# Autodesk Inventor assembly: Demonstrator
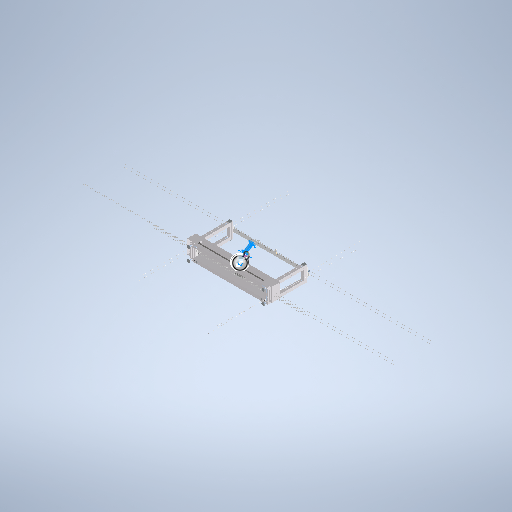
[picture p0: Inventor's stored thumbnail of the model, 512x512]
Saved by Autodesk Inventor 2025 (Build 290162010, 162A)
## iProperties
Created: 2024-11-07
Part Number: Demonstrator
Document SubType Name: Assembly
Designer: Admin
Mass: 19761.8 g
Surface Area: 23870.2 cm^2
Volume: 8041.77 cm^3
Density: 2.4574 g/cm^3
dummerWinkel: 1.5
Author: Admin
## Documents named in this file (25)
- C:\Users\Admin\GIT\HDVKBM\CAD\Krandemonstrator\Demonstrator.iam
- C:\Users\Admin\GIT\HDVKBM\CAD\Krandemonstrator\Träger.ipt
- C:\Users\Admin\Documents\Inventor\Content Center Files\R2025\de-DE\AS 1112 (2)\AS 1112 - M4  Typ 5.ipt
- C:\Users\Admin\GIT\HDVKBM\CAD\Krandemonstrator\MontageAufnahmeLO.ipt
- C:\Users\Admin\GIT\HDVKBM\CAD\Krandemonstrator\MontageAufnahmeLOV.ipt
- C:\Users\Admin\Documents\Inventor\Content Center Files\R2025\de-DE\AS 1427(03)\AS 1427 - M2 x 6(1).ipt
- C:\Users\Admin\GIT\HDVKBM\CAD\Krandemonstrator\Katze.iam
- C:\Users\Admin\GIT\HDVKBM\CAD\Krandemonstrator\UmlenkrolleHalterEinfach.iam
- C:\Users\Admin\GIT\HDVKBM\CAD\Krandemonstrator\SeilStange1m.ipt
- C:\Users\Admin\GIT\HDVKBM\CAD\Krandemonstrator\RollenhalterU.ipt
- C:\Users\Admin\GIT\HDVKBM\CAD\Krandemonstrator\UmlenkrolleHalterDoppelt.iam
- C:\Users\Admin\GIT\HDVKBM\CAD\Krandemonstrator\SeilatrappeHalter.ipt
- C:\Users\Admin\GIT\HDVKBM\CAD\Krandemonstrator\UmlenkrolleHalterDoppeltAngle.iam
- C:\Users\Admin\GIT\HDVKBM\CAD\Krandemonstrator\UmlenkrolleHalterEinfachAngle.iam
- C:\Users\Admin\GIT\HDVKBM\CAD\Krandemonstrator\UmlenkrolleHalterEinfachAngleB.iam
- C:\Users\Admin\GIT\HDVKBM\CAD\Krandemonstrator\seilatrappeHalterMini.ipt
- C:\Users\Admin\Documents\Inventor\Content Center Files\R2025\de-DE\AS 1421(4)\AS 1421 - M4 x 8 Kegelstumpf.ipt
- C:\Users\Admin\GIT\HDVKBM\CAD\Krandemonstrator\Schlitten.iam
- C:\Users\Admin\GIT\HDVKBM\CAD\Krandemonstrator\WS_10_40_930_2\WS_10_40_930_2.iam
- C:\Users\Admin\GIT\HDVKBM\CAD\Krandemonstrator\Frame.iam
- C:\Users\Admin\GIT\HDVKBM\CAD\Krandemonstrator\item_42006_nutenstein-8-st-m4-verzi__high\item_42006_nutenstein-8-st-m4-verzi__high.ipt
- C:\Users\Admin\Documents\Inventor\Content Center Files\R2025\de-DE\DIN 7991(2)\DIN 7991 - M4x30.ipt
- C:\Users\Admin\GIT\HDVKBM\CAD\Krandemonstrator\item_2623_nutenstein-8-st-m6-verzi__high\item_2623_nutenstein-8-st-m6-verzi__high.ipt
- C:\Users\Admin\Documents\Inventor\Content Center Files\R2025\de-DE\DIN 7991(2)\DIN 7991 - M6x16.ipt
- C:\Users\Admin\GIT\HDVKBM\CAD\Krandemonstrator\Zugfeder11.ipt
## Components (96 placed, 27 different names)
1. Katze:1 [sub-assembly] — KatzeLagerHO, KatzeLagerVV, KatzeSeilMutterVL, KatzeSeilMutterHL, KatzeSeilMutterVR, KatzeSeilMutterHR, KatzeGewindeSeilStumpfVL, KatzeGewindeSeilStumpfHL, KatzeGewindeSeilStumpfVR, KatzeGewindeSeilStumpfHR, KatzeSeilStumpfVL, KatzeSeilStumpfHL, KatzeSeilStumpfVR, KatzeSeilStumpfHR, Zylindrisch:83
2. Schlitten:1 [sub-assembly] — Verschiebbar:84, Zylindrisch:84, Zylindrisch:85, Zylindrisch:86, Zylindrisch:87, Planar:57, Planar:58, Planar:59, Planar:60
3. WS_10_40_930_2:1 [sub-assembly] — Zylindrisch:84, Zylindrisch:85, Zylindrisch:86, Zylindrisch:87, Starr:89, Starr:90, Starr:91, Starr:92, Starr:93, Starr:94, Starr:95, Starr:96, Starr:97
4. Frame:1 [sub-assembly] — Verschiebbar:85, Verschiebbar:86, Starr:83, Starr:88, Starr:89
5. item_42006_nutenstein-8-st-m4-verzi__high:1 — Starr:85
6. item_42006_nutenstein-8-st-m4-verzi__high:2 — Starr:84
7. item_42006_nutenstein-8-st-m4-verzi__high:3 — Starr:87
8. item_42006_nutenstein-8-st-m4-verzi__high:4 — Starr:86
9. DIN 7991 M4x30:1 — Passend:1
10. DIN 7991 M4x30:2 — Passend:2
11. DIN 7991 M4x30:3 — Passend:3
12. DIN 7991 M4x30:4 — Passend:4
13. DIN 7991 M6x16:1 — Starr:90, Starr:105
14. DIN 7991 M6x16:2 — Starr:91, Starr:104
15. DIN 7991 M6x16:3 — Starr:93, Starr:102
16. DIN 7991 M6x16:4 — Starr:92, Starr:103
17. DIN 7991 M6x16:5 — Starr:97, Starr:98
18. DIN 7991 M6x16:6 — Starr:96, Starr:99
19. DIN 7991 M6x16:7 — Starr:95, Starr:100
20. DIN 7991 M6x16:8 — Starr:94, Starr:101
21. item_2623_nutenstein-8-st-m6-verzi__high:1 — Starr:105
22. item_2623_nutenstein-8-st-m6-verzi__high:2 — Starr:104
23. item_2623_nutenstein-8-st-m6-verzi__high:3 — Starr:99
24. item_2623_nutenstein-8-st-m6-verzi__high:4 — Starr:103
25. item_2623_nutenstein-8-st-m6-verzi__high:5 — Starr:102
26. item_2623_nutenstein-8-st-m6-verzi__high:6 — Starr:101
27. item_2623_nutenstein-8-st-m6-verzi__high:7 — Starr:100
28. item_2623_nutenstein-8-st-m6-verzi__high:8 — Starr:98
29. Zugfeder1:1
30. MontageAufnahmeLOVV:2 — Starr:51, SeilrolleORHscrewA, SeilrolleORHscrewB, SeilrolleORHplan
31. MontageAufnahmeLO:2 — Starr:52, SeilrolleORVplan, SeilrolleORVscrewA, SeilrolleORVscrewB
32. MontageAufnahmeLOV:1 — SeilrolleOLVAuflage, SeilrolleOLVSchraubeA, SeilrolleOLVSchraubeB
33. MontageAufnahmeLOH:1 — SeilrolleOLHAuflage, SeilrolleOLHSchraubeA, SeilrolleOLHSchraubeB, Verschiebbar:85
34. Träger:1 — KatzeLagerHO, KatzeLagerVV, Starr:51, Starr:52, Verschiebbar:86
35. lastseil — Verschiebbar:84, Zylindrisch:83
36. seilatrappeHalterMini:3 — SeilAtrappeHalterMini3, SeilAtrappeHalterMini3Seil
37. seilatrappeHalterMini:4 — SeilAtrappeHalterMini4, SeilAtrappeHalterMini4Seil
38. SeilStange1m:16 — SeilrolleULMVsld, SeilAtrappeHalterMini3Seil, Planar:58
39. SeilStange1m:17 — SeilrolleULMHsld, SeilAtrappeHalterMini4Seil, Planar:57
40. SeilStange1m:18 — SeilAtrappeHalterMini1Seil, SeilrolleORVver, SeilrolleURMVver
41. SeilStange1m:19 — SeilAtrappeHalterMini2Seil, SeilrolleORHver, SeilrolleURMHver
42. seilatrappeHalterMini:1 — SeilAtrappeHalterMini1, SeilAtrappeHalterMini1Seil
43. seilatrappeHalterMini:2 — SeilAtrappeHalterMini2, SeilAtrappeHalterMini2Seil
44. SeilStange1m:13 — SeilrolleURHsld, Planar:59
45. SeilStange1m:12 — SeilrolleURVsld, Planar:60
46. SeilatrappeHalter:1 — SeilAtrappeHalterSeilA, SeilAtrappeHalterSeilB
47. SeilStange1m:1 — KatzeGewindeSeilStumpfVL, SeilrolleOLVhor
48. SeilStange1m:3 — SeilrolleOLHhor, KatzeSeilStumpfHL
49. SeilStange1m:4 — SeilrolleORHhor, KatzeSeilStumpfHR
50. SeilStange1m:5 — SeilrolleORVhor, KatzeSeilStumpfVR
51. SeilStange1m:8 — SeilAtrappeHalterSeilB, SeilrolleOLHver, SeilrolleULHver
52. SeilStange1m:9 — SeilAtrappeHalterSeilA, SeilrolleOLVver, SeilrolleULVver
53. SeilStange1m:10 — Zylindrisch:15, SeilrolleULHhor, SeilrolleURHhor
54. SeilStange1m:11 — Zylindrisch:16, SeilrolleULVhor, SeilrolleURVhor
55. SeilStange1m:14 — SeilAtrappeRollenhalterSeilB, SeilrolleULMHhor, SeilrolleURMHhor
56. SeilStange1m:15 — SeilAtrappeRollenhalterSeilA, SeilrolleULMVhor, SeilrolleURMVhor
57. AS 1427 - Metrisch M2 x 6:2 — SeilrolleOLVSchraube2, SeilrolleOLVSchraubeA
58. AS 1427 - Metrisch M2 x 6:1 — SeilrolleOLVSchraube1, SeilrolleOLVSchraubeB
59. UmlenkrolleHalterEinfach:1 [sub-assembly] — SeilrolleOLVSchraube1, SeilrolleOLVAuflage, SeilrolleOLVSchraube2, SeilrolleOLVhor, SeilrolleOLVver
60. AS 1427 - Metrisch M2 x 6:3 — SeilrolleOLHSchraube1, SeilrolleOLHSchraubeA
61. AS 1427 - Metrisch M2 x 6:4 — SeilrolleOLHSchraube2, SeilrolleOLHSchraubeB
62. UmlenkrolleHalterEinfach:2 [sub-assembly] — SeilrolleOLHSchraube1, SeilrolleOLHSchraube2, SeilrolleOLHAuflage, SeilrolleOLHhor, SeilrolleOLHver
63. AS 1112 (2) - Metrisch M4  Typ 5:4 — KatzeSeilMutterVR
64. AS 1112 (2) - Metrisch M4  Typ 5:3 — KatzeSeilMutterVL
65. AS 1112 (2) - Metrisch M4  Typ 5:2 — KatzeSeilMutterHR
66. AS 1112 (2) - Metrisch M4  Typ 5:1 — KatzeSeilMutterHL
67. AS 1421 Kegelstumpf - Metrisch M4 x 8 Kegelstumpf:4 — KatzeGewindeSeilStumpfHR
68. AS 1421 Kegelstumpf - Metrisch M4 x 8 Kegelstumpf:1 — KatzeGewindeSeilStumpfVR
69. AS 1421 Kegelstumpf - Metrisch M4 x 8 Kegelstumpf:2 — KatzeSeilStumpfVL
70. AS 1421 Kegelstumpf - Metrisch M4 x 8 Kegelstumpf:3 — KatzeGewindeSeilStumpfHL
71. UmlenkrolleHalterEinfachAngle:1 [sub-assembly] — SeilrolleORVscrewAfix, SeilrolleORVscrewBfix, SeilrolleORVplan, SeilrolleORVhor, SeilrolleORVver, SeilAtrappeHalterMini1
72. AS 1427 - Metrisch M2 x 6:17 — SeilrolleORVscrewBfix, SeilrolleORVscrewB
73. AS 1427 - Metrisch M2 x 6:18 — SeilrolleORVscrewAfix, SeilrolleORVscrewA
74. AS 1427 - Metrisch M2 x 6:19 — SeilrolleORHscrewB, SeilrolleORHscrewBfix
75. AS 1427 - Metrisch M2 x 6:20 — SeilrolleORHscrewA, SeilrolleORHscrewAfix
76. UmlenkrolleHalterEinfachAngleB:1 [sub-assembly] — SeilrolleORHplan, SeilrolleORHscrewAfix, SeilrolleORHscrewBfix, SeilAtrappeHalterMini2, SeilrolleORHhor, SeilrolleORHver
77. RollenhalterU:1 — Planar:24, Zylindrisch:5, Zylindrisch:6, Planar:25, Zylindrisch:7, Zylindrisch:8, Planar:40, Zylindrisch:9, Zylindrisch:10, Zylindrisch:15, Zylindrisch:16, Starr:84, Starr:85, Passend:1, Passend:2, Starr:88
78. UmlenkrolleHalterDoppelt:1 [sub-assembly] — Planar:24, Starr:33, Starr:34, SeilrolleULMHhor, SeilrolleULMVhor, SeilrolleULMHsld, SeilrolleULMVsld, SeilAtrappeHalterMini3, SeilAtrappeHalterMini4
79. UmlenkrolleHalterEinfach:3 [sub-assembly] — Starr:35, Starr:36, Planar:25, SeilrolleULVver, SeilrolleULVhor
80. UmlenkrolleHalterEinfach:4 [sub-assembly] — Starr:37, Starr:38, Planar:40, SeilrolleULHver, SeilrolleULHhor
81. AS 1427 - Metrisch M2 x 6:5 — Starr:38, Zylindrisch:9
82. AS 1427 - Metrisch M2 x 6:6 — Starr:37, Zylindrisch:10
83. AS 1427 - Metrisch M2 x 6:7 — Starr:34, Zylindrisch:6
84. AS 1427 - Metrisch M2 x 6:8 — Starr:33, Zylindrisch:5
85. AS 1427 - Metrisch M2 x 6:9 — Starr:35, Zylindrisch:8
86. AS 1427 - Metrisch M2 x 6:10 — Starr:36, Zylindrisch:7
87. UmlenkrolleHalterEinfach:5 [sub-assembly] — Starr:45, Starr:44, Planar:42, SeilrolleURVhor, SeilrolleURVsld
88. UmlenkrolleHalterEinfach:6 [sub-assembly] — Starr:46, Starr:47, Planar:43, SeilrolleURHhor, SeilrolleURHsld
89. UmlenkrolleHalterDoppeltAngle:1 [sub-assembly] — Planar:54, Starr:53, Starr:54, SeilrolleURMHhor, SeilrolleURMVhor, SeilrolleURMVver, SeilrolleURMHver
90. AS 1427 - Metrisch M2 x 6:11 — Starr:47, Zylindrisch:22
91. AS 1427 - Metrisch M2 x 6:12 — Starr:46, Zylindrisch:21
92. AS 1427 - Metrisch M2 x 6:13 — Starr:45, Zylindrisch:20
93. AS 1427 - Metrisch M2 x 6:14 — Zylindrisch:18, Starr:53
94. AS 1427 - Metrisch M2 x 6:15 — Zylindrisch:17, Starr:54
95. AS 1427 - Metrisch M2 x 6:16 — Starr:44, Zylindrisch:19
96. RollenhalterU:2 — Zylindrisch:17, Zylindrisch:18, Planar:42, Zylindrisch:19, Zylindrisch:20, Planar:43, Zylindrisch:21, Zylindrisch:22, Planar:54, SeilAtrappeRollenhalterSeilB, SeilAtrappeRollenhalterSeilA, Starr:83, Passend:3, Passend:4, Starr:86, Starr:87
## Relationships (143: WeldJoint 61, CylindricalJoint 35, RelateRotateTranslate 24, PlanarJoint 16, Mate 4, TranslationJoint 3)
- KatzeLagerHO [PlanarJoint] (0.05 mm): Katze:1 ↔ Träger:1
- KatzeLagerVV [PlanarJoint] (0.05 mm): Katze:1 ↔ Träger:1
- KatzeSeilMutterVL [WeldJoint]: Katze:1 ↔ AS 1112 (2) - Metrisch M4  Typ 5:3
- KatzeSeilMutterHL [WeldJoint]: Katze:1 ↔ AS 1112 (2) - Metrisch M4  Typ 5:1
- KatzeSeilMutterVR [WeldJoint]: Katze:1 ↔ AS 1112 (2) - Metrisch M4  Typ 5:4
- KatzeSeilMutterHR [WeldJoint]: Katze:1 ↔ AS 1112 (2) - Metrisch M4  Typ 5:2
- KatzeGewindeSeilStumpfVL [WeldJoint]: Katze:1 ↔ SeilStange1m:1
- KatzeGewindeSeilStumpfHL [WeldJoint]: Katze:1 ↔ AS 1421 Kegelstumpf - Metrisch M4 x 8 Kegelstumpf:3
- KatzeGewindeSeilStumpfVR [WeldJoint]: Katze:1 ↔ AS 1421 Kegelstumpf - Metrisch M4 x 8 Kegelstumpf:1
- KatzeGewindeSeilStumpfHR [WeldJoint]: Katze:1 ↔ AS 1421 Kegelstumpf - Metrisch M4 x 8 Kegelstumpf:4
- KatzeSeilStumpfVL [WeldJoint]: Katze:1 ↔ AS 1421 Kegelstumpf - Metrisch M4 x 8 Kegelstumpf:2
- KatzeSeilStumpfHL [WeldJoint]: Katze:1 ↔ SeilStange1m:3
- KatzeSeilStumpfVR [WeldJoint]: Katze:1 ↔ SeilStange1m:5
- KatzeSeilStumpfHR [WeldJoint]: Katze:1 ↔ SeilStange1m:4
- SeilrolleOLVSchraube1 [WeldJoint]: AS 1427 - Metrisch M2 x 6:1 ↔ UmlenkrolleHalterEinfach:1
- SeilrolleOLVSchraube2 [WeldJoint]: AS 1427 - Metrisch M2 x 6:2 ↔ UmlenkrolleHalterEinfach:1
- SeilrolleOLVAuflage [PlanarJoint]: MontageAufnahmeLOV:1 ↔ UmlenkrolleHalterEinfach:1
- SeilrolleOLVSchraubeA [CylindricalJoint]: MontageAufnahmeLOV:1 ↔ AS 1427 - Metrisch M2 x 6:2
- SeilrolleOLVSchraubeB [CylindricalJoint]: MontageAufnahmeLOV:1 ↔ AS 1427 - Metrisch M2 x 6:1
- SeilrolleOLVhor [RelateRotateTranslate] (9 mm): SeilStange1m:1 ↔ UmlenkrolleHalterEinfach:1
- SeilrolleOLVver [RelateRotateTranslate] (9 mm): SeilStange1m:9 ↔ UmlenkrolleHalterEinfach:1
- SeilrolleOLHSchraube1 [WeldJoint]: AS 1427 - Metrisch M2 x 6:3 ↔ UmlenkrolleHalterEinfach:2
- SeilrolleOLHSchraube2 [WeldJoint]: AS 1427 - Metrisch M2 x 6:4 ↔ UmlenkrolleHalterEinfach:2
- SeilrolleOLHAuflage [PlanarJoint]: MontageAufnahmeLOH:1 ↔ UmlenkrolleHalterEinfach:2
- SeilrolleOLHSchraubeA [CylindricalJoint]: MontageAufnahmeLOH:1 ↔ AS 1427 - Metrisch M2 x 6:3
- SeilrolleOLHSchraubeB [CylindricalJoint]: MontageAufnahmeLOH:1 ↔ AS 1427 - Metrisch M2 x 6:4
- SeilrolleOLHhor [RelateRotateTranslate] (9 mm): SeilStange1m:3 ↔ UmlenkrolleHalterEinfach:2
- SeilrolleOLHver [RelateRotateTranslate] (9 mm): SeilStange1m:8 ↔ UmlenkrolleHalterEinfach:2
- Planar:24: RollenhalterU:1 ↔ UmlenkrolleHalterDoppelt:1
- Starr:33 [WeldJoint]: UmlenkrolleHalterDoppelt:1 ↔ AS 1427 - Metrisch M2 x 6:8
- Starr:34 [WeldJoint]: UmlenkrolleHalterDoppelt:1 ↔ AS 1427 - Metrisch M2 x 6:7
- Zylindrisch:5 [CylindricalJoint]: RollenhalterU:1 ↔ AS 1427 - Metrisch M2 x 6:8
- Zylindrisch:6 [CylindricalJoint]: RollenhalterU:1 ↔ AS 1427 - Metrisch M2 x 6:7
- Starr:35 [WeldJoint]: UmlenkrolleHalterEinfach:3 ↔ AS 1427 - Metrisch M2 x 6:9
- Starr:36 [WeldJoint]: UmlenkrolleHalterEinfach:3 ↔ AS 1427 - Metrisch M2 x 6:10
- Planar:25: RollenhalterU:1 ↔ UmlenkrolleHalterEinfach:3
- Zylindrisch:7 [CylindricalJoint]: RollenhalterU:1 ↔ AS 1427 - Metrisch M2 x 6:10
- Zylindrisch:8 [CylindricalJoint]: RollenhalterU:1 ↔ AS 1427 - Metrisch M2 x 6:9
- Starr:37 [WeldJoint]: UmlenkrolleHalterEinfach:4 ↔ AS 1427 - Metrisch M2 x 6:6
- Starr:38 [WeldJoint]: UmlenkrolleHalterEinfach:4 ↔ AS 1427 - Metrisch M2 x 6:5
- Planar:40: RollenhalterU:1 ↔ UmlenkrolleHalterEinfach:4
- Zylindrisch:9 [CylindricalJoint]: RollenhalterU:1 ↔ AS 1427 - Metrisch M2 x 6:5
- Zylindrisch:10 [CylindricalJoint]: RollenhalterU:1 ↔ AS 1427 - Metrisch M2 x 6:6
- SeilAtrappeHalterSeilA [CylindricalJoint]: SeilatrappeHalter:1 ↔ SeilStange1m:9
- SeilAtrappeHalterSeilB [CylindricalJoint]: SeilatrappeHalter:1 ↔ SeilStange1m:8
- Zylindrisch:15 [CylindricalJoint]: SeilStange1m:10 ↔ RollenhalterU:1
- Zylindrisch:16 [CylindricalJoint]: SeilStange1m:11 ↔ RollenhalterU:1
- SeilrolleULVver [RelateRotateTranslate] (9 mm): SeilStange1m:9 ↔ UmlenkrolleHalterEinfach:3
- SeilrolleULHver [RelateRotateTranslate] (9 mm): SeilStange1m:8 ↔ UmlenkrolleHalterEinfach:4
- SeilrolleULVhor [RelateRotateTranslate] (9 mm): SeilStange1m:11 ↔ UmlenkrolleHalterEinfach:3
- SeilrolleULHhor [RelateRotateTranslate] (9 mm): SeilStange1m:10 ↔ UmlenkrolleHalterEinfach:4
- Zylindrisch:17 [CylindricalJoint]: AS 1427 - Metrisch M2 x 6:15 ↔ RollenhalterU:2
- Zylindrisch:18 [CylindricalJoint]: AS 1427 - Metrisch M2 x 6:14 ↔ RollenhalterU:2
- Starr:45 [WeldJoint]: UmlenkrolleHalterEinfach:5 ↔ AS 1427 - Metrisch M2 x 6:13
- Starr:44 [WeldJoint]: UmlenkrolleHalterEinfach:5 ↔ AS 1427 - Metrisch M2 x 6:16
- Planar:42: UmlenkrolleHalterEinfach:5 ↔ RollenhalterU:2
- Zylindrisch:19 [CylindricalJoint]: AS 1427 - Metrisch M2 x 6:16 ↔ RollenhalterU:2
- Zylindrisch:20 [CylindricalJoint]: AS 1427 - Metrisch M2 x 6:13 ↔ RollenhalterU:2
- Starr:46 [WeldJoint]: UmlenkrolleHalterEinfach:6 ↔ AS 1427 - Metrisch M2 x 6:12
- Starr:47 [WeldJoint]: UmlenkrolleHalterEinfach:6 ↔ AS 1427 - Metrisch M2 x 6:11
- Planar:43: UmlenkrolleHalterEinfach:6 ↔ RollenhalterU:2
- Zylindrisch:21 [CylindricalJoint]: AS 1427 - Metrisch M2 x 6:12 ↔ RollenhalterU:2
- Zylindrisch:22 [CylindricalJoint]: AS 1427 - Metrisch M2 x 6:11 ↔ RollenhalterU:2
- SeilrolleURHhor [RelateRotateTranslate] (9 mm): SeilStange1m:10 ↔ UmlenkrolleHalterEinfach:6
- SeilrolleURVhor [RelateRotateTranslate] (9 mm): SeilStange1m:11 ↔ UmlenkrolleHalterEinfach:5
- SeilrolleURVsld [RelateRotateTranslate] (9 mm): SeilStange1m:12 ↔ UmlenkrolleHalterEinfach:5
- SeilrolleURHsld [RelateRotateTranslate] (9 mm): SeilStange1m:13 ↔ UmlenkrolleHalterEinfach:6
- Starr:51 [WeldJoint]: MontageAufnahmeLOVV:2 ↔ Träger:1
- Starr:52 [WeldJoint]: MontageAufnahmeLO:2 ↔ Träger:1
- Planar:54: UmlenkrolleHalterDoppeltAngle:1 ↔ RollenhalterU:2
- Starr:53 [WeldJoint]: UmlenkrolleHalterDoppeltAngle:1 ↔ AS 1427 - Metrisch M2 x 6:14
- Starr:54 [WeldJoint]: UmlenkrolleHalterDoppeltAngle:1 ↔ AS 1427 - Metrisch M2 x 6:15
- SeilrolleORVscrewAfix [WeldJoint]: UmlenkrolleHalterEinfachAngle:1 ↔ AS 1427 - Metrisch M2 x 6:18
- SeilrolleORVscrewBfix [WeldJoint]: UmlenkrolleHalterEinfachAngle:1 ↔ AS 1427 - Metrisch M2 x 6:17
- SeilrolleORVplan [PlanarJoint]: MontageAufnahmeLO:2 ↔ UmlenkrolleHalterEinfachAngle:1
- SeilrolleORVscrewA [CylindricalJoint]: MontageAufnahmeLO:2 ↔ AS 1427 - Metrisch M2 x 6:18
- SeilrolleORVscrewB [CylindricalJoint]: MontageAufnahmeLO:2 ↔ AS 1427 - Metrisch M2 x 6:17
- SeilrolleORHscrewA [CylindricalJoint]: MontageAufnahmeLOVV:2 ↔ AS 1427 - Metrisch M2 x 6:20
- SeilrolleORHscrewB [CylindricalJoint]: MontageAufnahmeLOVV:2 ↔ AS 1427 - Metrisch M2 x 6:19
- SeilrolleORHplan [PlanarJoint]: MontageAufnahmeLOVV:2 ↔ UmlenkrolleHalterEinfachAngleB:1
- SeilrolleORHscrewAfix [WeldJoint]: AS 1427 - Metrisch M2 x 6:20 ↔ UmlenkrolleHalterEinfachAngleB:1
- SeilrolleORHscrewBfix [WeldJoint]: AS 1427 - Metrisch M2 x 6:19 ↔ UmlenkrolleHalterEinfachAngleB:1
- SeilAtrappeRollenhalterSeilB [CylindricalJoint]: SeilStange1m:14 ↔ RollenhalterU:2
- SeilAtrappeRollenhalterSeilA [CylindricalJoint]: SeilStange1m:15 ↔ RollenhalterU:2
- SeilrolleORHhor [RelateRotateTranslate] (9 mm): SeilStange1m:4 ↔ UmlenkrolleHalterEinfachAngleB:1
- SeilrolleORVhor [RelateRotateTranslate] (9 mm): SeilStange1m:5 ↔ UmlenkrolleHalterEinfachAngle:1
- SeilrolleORHver [RelateRotateTranslate] (9 mm): SeilStange1m:19 ↔ UmlenkrolleHalterEinfachAngleB:1
- SeilrolleORVver [RelateRotateTranslate] (9 mm): SeilStange1m:18 ↔ UmlenkrolleHalterEinfachAngle:1
- SeilrolleURMHhor [RelateRotateTranslate] (9 mm): SeilStange1m:14 ↔ UmlenkrolleHalterDoppeltAngle:1
- SeilrolleURMVhor [RelateRotateTranslate] (9 mm): SeilStange1m:15 ↔ UmlenkrolleHalterDoppeltAngle:1
- SeilrolleURMVver [RelateRotateTranslate] (9 mm): SeilStange1m:18 ↔ UmlenkrolleHalterDoppeltAngle:1
- SeilrolleURMHver [RelateRotateTranslate] (9 mm): SeilStange1m:19 ↔ UmlenkrolleHalterDoppeltAngle:1
- SeilrolleULMHhor [RelateRotateTranslate] (9 mm): SeilStange1m:14 ↔ UmlenkrolleHalterDoppelt:1
- SeilrolleULMVhor [RelateRotateTranslate] (9 mm): SeilStange1m:15 ↔ UmlenkrolleHalterDoppelt:1
- SeilrolleULMHsld [RelateRotateTranslate] (9 mm): SeilStange1m:17 ↔ UmlenkrolleHalterDoppelt:1
- SeilrolleULMVsld [RelateRotateTranslate] (9 mm): SeilStange1m:16 ↔ UmlenkrolleHalterDoppelt:1
- SeilAtrappeHalterMini1 [WeldJoint]: seilatrappeHalterMini:1 ↔ UmlenkrolleHalterEinfachAngle:1
- SeilAtrappeHalterMini1Seil [CylindricalJoint]: SeilStange1m:18 ↔ seilatrappeHalterMini:1
- SeilAtrappeHalterMini2 [WeldJoint]: seilatrappeHalterMini:2 ↔ UmlenkrolleHalterEinfachAngleB:1
- SeilAtrappeHalterMini2Seil [CylindricalJoint]: SeilStange1m:19 ↔ seilatrappeHalterMini:2
- SeilAtrappeHalterMini3 [WeldJoint]: seilatrappeHalterMini:3 ↔ UmlenkrolleHalterDoppelt:1
- SeilAtrappeHalterMini3Seil [CylindricalJoint]: seilatrappeHalterMini:3 ↔ SeilStange1m:16
- SeilAtrappeHalterMini4 [WeldJoint]: seilatrappeHalterMini:4 ↔ UmlenkrolleHalterDoppelt:1
- SeilAtrappeHalterMini4Seil [CylindricalJoint]: seilatrappeHalterMini:4 ↔ SeilStange1m:17
- Verschiebbar:84 [TranslationJoint]: Schlitten:1 ↔ lastseil
- Zylindrisch:83 [CylindricalJoint]: Katze:1 ↔ lastseil
- Zylindrisch:84 [CylindricalJoint]: Schlitten:1 ↔ WS_10_40_930_2:1
- Zylindrisch:85 [CylindricalJoint]: Schlitten:1 ↔ WS_10_40_930_2:1
- Zylindrisch:86 [CylindricalJoint]: Schlitten:1 ↔ WS_10_40_930_2:1
- Zylindrisch:87 [CylindricalJoint]: Schlitten:1 ↔ WS_10_40_930_2:1
- Planar:57 (-20 mm): Schlitten:1 ↔ SeilStange1m:17
- Planar:58 (-20 mm): Schlitten:1 ↔ SeilStange1m:16
- Planar:59 (-20 mm): Schlitten:1 ↔ SeilStange1m:13
- Planar:60 (-20 mm): Schlitten:1 ↔ SeilStange1m:12
- Verschiebbar:85 [TranslationJoint]: Frame:1 ↔ MontageAufnahmeLOH:1
- Verschiebbar:86 [TranslationJoint]: Frame:1 ↔ Träger:1
- Starr:83 [WeldJoint]: Frame:1 ↔ RollenhalterU:2
- Starr:84 [WeldJoint]: item_42006_nutenstein-8-st-m4-verzi__high:2 ↔ RollenhalterU:1
- Starr:85 [WeldJoint]: item_42006_nutenstein-8-st-m4-verzi__high:1 ↔ RollenhalterU:1
- Passend:1 [Mate]: DIN 7991 M4x30:1 ↔ RollenhalterU:1
- Passend:2 [Mate]: DIN 7991 M4x30:2 ↔ RollenhalterU:1
- Passend:3 [Mate]: DIN 7991 M4x30:3 ↔ RollenhalterU:2
- Passend:4 [Mate]: DIN 7991 M4x30:4 ↔ RollenhalterU:2
- Starr:86 [WeldJoint]: item_42006_nutenstein-8-st-m4-verzi__high:4 ↔ RollenhalterU:2
- Starr:87 [WeldJoint]: item_42006_nutenstein-8-st-m4-verzi__high:3 ↔ RollenhalterU:2
- Starr:88 [WeldJoint]: Frame:1 ↔ RollenhalterU:1
- Starr:89 [WeldJoint] (1.5 mm): WS_10_40_930_2:1 ↔ Frame:1
- Starr:90 [WeldJoint]: WS_10_40_930_2:1 ↔ DIN 7991 M6x16:1
- Starr:91 [WeldJoint]: WS_10_40_930_2:1 ↔ DIN 7991 M6x16:2
- Starr:92 [WeldJoint]: WS_10_40_930_2:1 ↔ DIN 7991 M6x16:4
- Starr:93 [WeldJoint]: WS_10_40_930_2:1 ↔ DIN 7991 M6x16:3
- Starr:94 [WeldJoint]: WS_10_40_930_2:1 ↔ DIN 7991 M6x16:8
- Starr:95 [WeldJoint]: WS_10_40_930_2:1 ↔ DIN 7991 M6x16:7
- Starr:96 [WeldJoint]: WS_10_40_930_2:1 ↔ DIN 7991 M6x16:6
- Starr:97 [WeldJoint]: WS_10_40_930_2:1 ↔ DIN 7991 M6x16:5
- Starr:98 [WeldJoint]: DIN 7991 M6x16:5 ↔ item_2623_nutenstein-8-st-m6-verzi__high:8
- Starr:99 [WeldJoint]: DIN 7991 M6x16:6 ↔ item_2623_nutenstein-8-st-m6-verzi__high:3
- Starr:100 [WeldJoint]: DIN 7991 M6x16:7 ↔ item_2623_nutenstein-8-st-m6-verzi__high:7
- Starr:101 [WeldJoint]: DIN 7991 M6x16:8 ↔ item_2623_nutenstein-8-st-m6-verzi__high:6
- Starr:102 [WeldJoint]: DIN 7991 M6x16:3 ↔ item_2623_nutenstein-8-st-m6-verzi__high:5
- Starr:103 [WeldJoint]: DIN 7991 M6x16:4 ↔ item_2623_nutenstein-8-st-m6-verzi__high:4
- Starr:104 [WeldJoint]: DIN 7991 M6x16:2 ↔ item_2623_nutenstein-8-st-m6-verzi__high:2
- Starr:105 [WeldJoint]: DIN 7991 M6x16:1 ↔ item_2623_nutenstein-8-st-m6-verzi__high:1
## Named parameters: Finish2_Area = 2136.28, Finish3_Area = 43.5425, Finish4_Area = 0.0628319
note: some values were not read from the file. Shown as the stored number, unit unknown: "Finish2_Area", "Finish3_Area", "Finish4_Area".
